# Autodesk Inventor assembly: zlozenieTymRazemOdwrotniezUchwytem
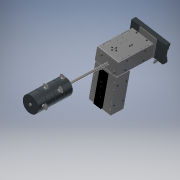
[picture p0: Inventor's stored thumbnail of the model, 180x180]
Saved by Autodesk Inventor 2019 (Build 230136000, 136)
## iProperties
Created: 2020-08-29
Part Number: zlozenieTymRazemOdwrotniezUchwytem
Document SubType Name: Assembly
Designer: estee
Author: estee
## Documents named in this file (15)
- C:\Users\estee\OneDrive\Pulpit\estere\1\MUM\wogoleNajnowszyGit\Mechanika\Moduł obrotu RET Estera\prawieKoncowka\zlozenieTymRazemOdwrotniezUchwytem.iam
- C:\Users\estee\OneDrive\Pulpit\estere\1\MUM\wogoleNajnowszyGit\Mechanika\Moduł obrotu RET Estera\prawieKoncowka\ObudowaNowa.iam
- C:\Users\estee\OneDrive\Pulpit\estere\1\MUM\wogoleNajnowszyGit\Mechanika\Moduł obrotu RET Estera\prawieKoncowka\ObudowaNowa2.iam
- C:\Users\estee\OneDrive\Pulpit\estere\1\MUM\wogoleNajnowszyGit\Mechanika\Moduł obrotu RET Estera\prawieKoncowka\ISO 4026 - M3 x 3 - ISO.ipt
- C:\Users\estee\OneDrive\Pulpit\estere\1\MUM\wogoleNajnowszyGit\Mechanika\Moduł obrotu RET Estera\prawieKoncowka\trzymak.iam
- C:\Users\estee\OneDrive\Pulpit\estere\1\MUM\wogoleNajnowszyGit\Mechanika\Moduł obrotu RET Estera\prawieKoncowka\dovetail.ipt
- C:\Users\estee\OneDrive\Pulpit\estere\1\MUM\wogoleNajnowszyGit\Mechanika\Moduł obrotu RET Estera\prawieKoncowka\Połączenie gwintowe1.iam
- C:\Users\estee\OneDrive\Pulpit\estere\1\MUM\wogoleNajnowszyGit\Mechanika\Moduł obrotu RET Estera\prawieKoncowka\Połączenie gwintowe2.iam
- C:\Users\estee\OneDrive\Pulpit\estere\1\MUM\wogoleNajnowszyGit\Mechanika\Moduł obrotu RET Estera\prawieKoncowka\Połączenie gwintowe4.iam
- F:\GOTOWY BEM\PRIMATYMIRROR\Połączenie gwintowe5.iam
- F:\GOTOWY BEM\PRIMATYMIRROR\Połączenie gwintowe6.iam
- F:\GOTOWY BEM\PRIMATYMIRROR\Połączenie gwintowe7.iam
- C:\Users\estee\OneDrive\Pulpit\estere\1\MUM\wogoleNajnowszyGit\Mechanika\Moduł obrotu RET Estera\prawieKoncowka\Połączenie gwintowe8.iam
- C:\Users\estee\OneDrive\Pulpit\estere\1\MUM\wogoleNajnowszyGit\Mechanika\Moduł obrotu RET Estera\prawieKoncowka\Połączenie gwintowe9.iam
- C:\Users\estee\OneDrive\Pulpit\estere\1\MUM\wogoleNajnowszyGit\Mechanika\Moduł obrotu RET Estera\prawieKoncowka\ciezarekztytkiem.iam
## Components (22 placed, 7 different names)
1. ObudowaNowa:1 [sub-assembly] — Angle:1, Tangent:1, Tangent:2, Tangent:3, Tangent:4, Mate:14, Mate:15, Zestawiające:16, Zestawiające:17, Zestawiające:18
2. ObudowaNowa2:1 [sub-assembly] — Angle:1, Mate:3, Mate:4, Mate:5, Mate:6, Mate:7, Mate:8, Angle:2, Tangent:5, Tangent:6, Mate:13, Mate:14, Mate:15, Mate:67, Mate:68, Mate:69, Mate:70, Flush:1
3. ISO 4026 M3 x 3:1 — Mate:7, Tangent:4
4. ISO 4026 M3 x 3:2 — Mate:5, Tangent:3
5. ISO 4026 M3 x 3:3 — Mate:3, Mate:6, Tangent:1
6. ISO 4026 M3 x 3:4 — Mate:4, Tangent:2
7. trzymak:1 [sub-assembly] — Mate:8, Angle:2, Mate:11, Mate:12, Mate:13
8. ISO 4026 M3 x 3:5 — Mate:11, Tangent:5
9. ISO 4026 M3 x 3:6 — Mate:12, Tangent:6
10. dovetail:1 — Zestawiające:16, Zestawiające:17, Zestawiające:18, Zestawiające:19, Zestawiające:20, Zestawiające:21, Zestawiające:22, Zestawiające:23, Zestawiające:24, Zestawiające:25, Zestawiające:26, Zestawiające:27, Zestawiające:28, Zestawiające:29, Zestawiające:30, Zestawiające:31, Zestawiające:32, Zestawiające:33, Zestawiające:34
11. Połączenie gwintowe:1 [sub-assembly] — Zestawiające:19, Zestawiające:20
12. Połączenie gwintowe:2 [sub-assembly] — Zestawiające:21, Zestawiające:22
13. Połączenie gwintowe:3 [sub-assembly] — Zestawiające:23, Zestawiające:24
14. Połączenie gwintowe:4 [sub-assembly] — Zestawiające:25, Zestawiające:26
15. Połączenie gwintowe:5 [sub-assembly] — Zestawiające:27, Zestawiające:28
16. Połączenie gwintowe:6 [sub-assembly] — Zestawiające:29, Zestawiające:30
17. Połączenie gwintowe:7 [sub-assembly] — Zestawiające:31, Zestawiające:32
18. Połączenie gwintowe:8 [sub-assembly] — Zestawiające:33, Zestawiające:34
19. ciezarekztytkiem:1 [sub-assembly] — Mate:67, Mate:72, Mate:73
20. ciezarekztytkiem:2 [sub-assembly] — Mate:70, Mate:73
21. ciezarekztytkiem:3 [sub-assembly] — Mate:68, Mate:71, Mate:72
22. ciezarekztytkiem:4 [sub-assembly] — Mate:69, Flush:1, Mate:71
## Relationships (46: Mate 37, Tangent 6, Angle 2, Flush 1)
- Angle:1 (0 deg): ObudowaNowa:1 ↔ ObudowaNowa2:1
- Mate:3: ObudowaNowa2:1 ↔ ISO 4026 M3 x 3:3
- Mate:4: ObudowaNowa2:1 ↔ ISO 4026 M3 x 3:4
- Mate:5: ObudowaNowa2:1 ↔ ISO 4026 M3 x 3:2
- Mate:6: ObudowaNowa2:1 ↔ ISO 4026 M3 x 3:3
- Tangent:1: ObudowaNowa:1 ↔ ISO 4026 M3 x 3:3
- Tangent:2: ObudowaNowa:1 ↔ ISO 4026 M3 x 3:4
- Tangent:3: ObudowaNowa:1 ↔ ISO 4026 M3 x 3:2
- Mate:7: ObudowaNowa2:1 ↔ ISO 4026 M3 x 3:1
- Tangent:4: ObudowaNowa:1 ↔ ISO 4026 M3 x 3:1
- Mate:8: ObudowaNowa2:1 ↔ trzymak:1
- Angle:2 (0 deg): ObudowaNowa2:1 ↔ trzymak:1
- Mate:11: trzymak:1 ↔ ISO 4026 M3 x 3:5
- Tangent:5: ObudowaNowa2:1 ↔ ISO 4026 M3 x 3:5
- Mate:12: trzymak:1 ↔ ISO 4026 M3 x 3:6
- Tangent:6: ObudowaNowa2:1 ↔ ISO 4026 M3 x 3:6
- Mate:13: ObudowaNowa2:1 ↔ trzymak:1
- Mate:14: ObudowaNowa:1 ↔ ObudowaNowa2:1
- Mate:15 (10 mm): ObudowaNowa:1 ↔ ObudowaNowa2:1
- Zestawiające:16 [Mate]: ObudowaNowa:1 ↔ dovetail:1
- Zestawiające:17 [Mate]: ObudowaNowa:1 ↔ dovetail:1
- Zestawiające:18 [Mate]: ObudowaNowa:1 ↔ dovetail:1
- Zestawiające:19 [Mate]: dovetail:1 ↔ Połączenie gwintowe:1
- Zestawiające:20 [Mate]: dovetail:1 ↔ Połączenie gwintowe:1
- Zestawiające:21 [Mate]: dovetail:1 ↔ Połączenie gwintowe:2
- Zestawiające:22 [Mate]: dovetail:1 ↔ Połączenie gwintowe:2
- Zestawiające:23 [Mate]: dovetail:1 ↔ Połączenie gwintowe:3
- Zestawiające:24 [Mate]: dovetail:1 ↔ Połączenie gwintowe:3
- Zestawiające:25 [Mate]: dovetail:1 ↔ Połączenie gwintowe:4
- Zestawiające:26 [Mate]: dovetail:1 ↔ Połączenie gwintowe:4
- Zestawiające:27 [Mate]: dovetail:1 ↔ Połączenie gwintowe:5
- Zestawiające:28 [Mate]: dovetail:1 ↔ Połączenie gwintowe:5
- Zestawiające:29 [Mate]: dovetail:1 ↔ Połączenie gwintowe:6
- Zestawiające:30 [Mate]: dovetail:1 ↔ Połączenie gwintowe:6
- Zestawiające:31 [Mate]: dovetail:1 ↔ Połączenie gwintowe:7
- Zestawiające:32 [Mate]: dovetail:1 ↔ Połączenie gwintowe:7
- Zestawiające:33 [Mate]: dovetail:1 ↔ Połączenie gwintowe:8
- Zestawiające:34 [Mate]: dovetail:1 ↔ Połączenie gwintowe:8
- Mate:67: ObudowaNowa2:1 ↔ ciezarekztytkiem:1
- Mate:68: ObudowaNowa2:1 ↔ ciezarekztytkiem:3
- Mate:69: ObudowaNowa2:1 ↔ ciezarekztytkiem:4
- Mate:70: ObudowaNowa2:1 ↔ ciezarekztytkiem:2
- Flush:1 (5 mm): ObudowaNowa2:1 ↔ ciezarekztytkiem:4
- Mate:71: ciezarekztytkiem:3 ↔ ciezarekztytkiem:4
- Mate:72: ciezarekztytkiem:1 ↔ ciezarekztytkiem:3
- Mate:73: ciezarekztytkiem:1 ↔ ciezarekztytkiem:2
